# Autodesk Inventor assembly: Rear Worm Drive_MIR
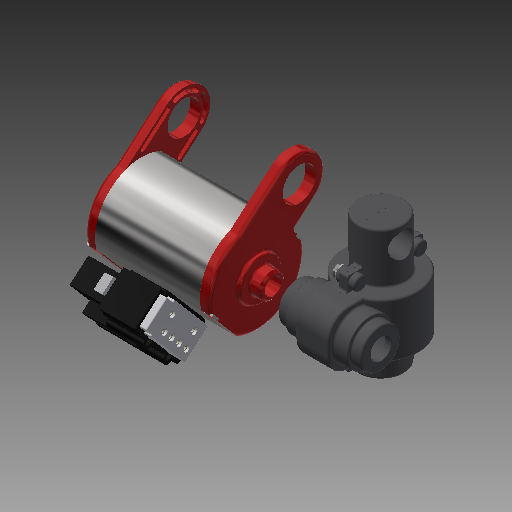
[picture p0: Inventor's stored thumbnail of the model, 512x512]
Saved by Autodesk Inventor 2019 (Build 230136000, 136)
## iProperties
Company: Autodesk Inc.
Created: 2008-01-21
Part Number: Rear Worm Drive_MIR
Document SubType Name: Assembly
Designer: Autodesk Inc.
Mass: 126.589 g
Surface Area: 610.96 cm^2
Volume: 70.4052 cm^3
Density: 1.798 g/cm^3
Author: Inventor
## Documents named in this file (5)
- C:\TEMP\Car Seat\Workspace\Rear Worm Drive_MIR.iam
- C:\TEMP\Car Seat\Workspace\AS 1417 - Metric M3 x 6.ipt
- C:\TEMP\Car Seat\Workspace\Motor.iam
- C:\TEMP\Car Seat\Workspace\Rear Worm Casing L.ipt
- C:\TEMP\Car Seat\Workspace\Rear Worm Casing R.ipt
## Components (7 placed, 4 different names)
1. Rear Worm Casing R:1 — Mate:12, Mate:3, Mate:1, Mate:11, Mate:10
2. AS 1427 - Metric M3 x 6:1 — Insert:1
3. AS 1427 - Metric M3 x 6:2 — Insert:2
4. AS 1427 - Metric M3 x 6:3 — Insert:3
5. AS 1427 - Metric M3 x 6:4 — Insert:4
6. Rear Worm Casing L:1 — Mate:12, Mate:3, Mate:1, Mate:13, Insert:1, Insert:2, Insert:3, Insert:4
7. Motor:1 [sub-assembly] — Mate:13, Mate:11, Mate:10
## Relationships (10: Mate 6, Insert 4)
- Mate:12: Rear Worm Casing R:1 ↔ Rear Worm Casing L:1
- Mate:3: Rear Worm Casing R:1 ↔ Rear Worm Casing L:1
- Mate:1: Rear Worm Casing R:1 ↔ Rear Worm Casing L:1
- Insert:1: AS 1427 - Metric M3 x 6:1 ↔ Rear Worm Casing L:1
- Insert:2: AS 1427 - Metric M3 x 6:2 ↔ Rear Worm Casing L:1
- Insert:3: AS 1427 - Metric M3 x 6:3 ↔ Rear Worm Casing L:1
- Insert:4: AS 1427 - Metric M3 x 6:4 ↔ Rear Worm Casing L:1
- Mate:13 (11.5 mm): Rear Worm Casing L:1 ↔ Motor:1
- Mate:11: Rear Worm Casing R:1 ↔ Motor:1
- Mate:10: Rear Worm Casing R:1 ↔ Motor:1
